# Autodesk Inventor assembly: Assembly1
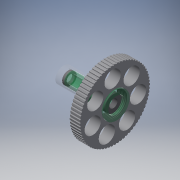
[picture p0: Inventor's stored thumbnail of the model, 180x180]
Saved by Autodesk Inventor 2018.1 (Build 221171000, 171)
## iProperties
Created: 2022-06-29
Part Number: Assembly1
Document SubType Name: Assembly
Designer: Bureau
Author: Bureau
## Documents named in this file (6)
- C:\Users\Bureau\Mon Drive\Manu\USINAGE\MoteurVelo\Arbre secondaire\Assembly1.iam
- C:\Users\Bureau\Mon Drive\Manu\USINAGE\MoteurVelo\Arbre secondaire\bague 12 x16 x23.ipt
- C:\Users\Bureau\Mon Drive\Manu\USINAGE\MoteurVelo\Arbre secondaire\entraineur poulie 72.ipt
- C:\Users\Bureau\Mon Drive\Manu\USINAGE\MoteurVelo\Arbre secondaire\roulement 8 x 12 x 2.5.ipt
- C:\Users\Bureau\Mon Drive\Manu\USINAGE\MoteurVelo\Arbre secondaire\roulement 8 x 16 x 5.ipt
- C:\Users\Bureau\Mon Drive\Manu\USINAGE\MoteurVelo\Arbre secondaire\poulie 72 dents.ipt
## Components (6 placed, 5 different names)
1. bague 12 x16 x23:1 — Mate:3, Mate:9, Mate:13, Mate:14
2. entraineur poulie 72:1 — Mate:4, Mate:5, Mate:7, Mate:10, Mate:12, Mate:13, Mate:14
3. roulement 8 x 12 x 2.5:1 — Mate:3, Mate:4, Mate:12
4. roulement 8 x 16 x 5:1 — Mate:5, Mate:6, Mate:11
5. roulement 8 x 16 x 5:2 — Mate:6, Mate:7, Mate:11
6. poulie 72 dents:1 — Mate:9, Mate:10
## Relationships (11: Mate 11)
- Mate:3: bague 12 x16 x23:1 ↔ roulement 8 x 12 x 2.5:1
- Mate:4: entraineur poulie 72:1 ↔ roulement 8 x 12 x 2.5:1
- Mate:5: entraineur poulie 72:1 ↔ roulement 8 x 16 x 5:1
- Mate:6: roulement 8 x 16 x 5:1 ↔ roulement 8 x 16 x 5:2
- Mate:7: entraineur poulie 72:1 ↔ roulement 8 x 16 x 5:2
- Mate:9: bague 12 x16 x23:1 ↔ poulie 72 dents:1
- Mate:10: entraineur poulie 72:1 ↔ poulie 72 dents:1
- Mate:11 (14 mm): roulement 8 x 16 x 5:1 ↔ roulement 8 x 16 x 5:2
- Mate:12: entraineur poulie 72:1 ↔ roulement 8 x 12 x 2.5:1
- Mate:13: bague 12 x16 x23:1 ↔ entraineur poulie 72:1
- Mate:14: bague 12 x16 x23:1 ↔ entraineur poulie 72:1
